# Autodesk Inventor assembly: Back_Panel_Assembly
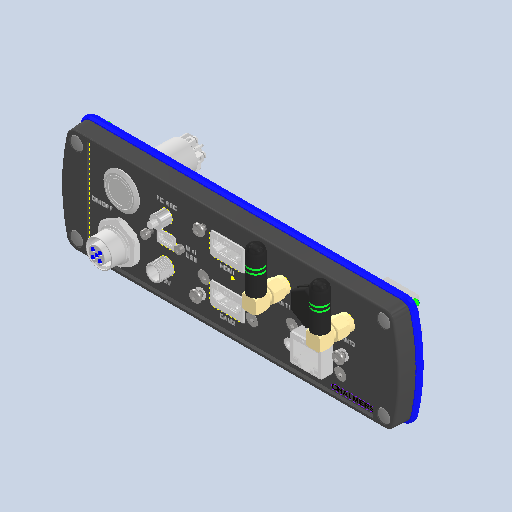
[picture p0: Inventor's stored thumbnail of the model, 512x512]
Saved by Autodesk Inventor 2022 (Build 260153000, 153)
## iProperties
Created: 2020-07-14
Part Number: Back_Panel_Assembly
Document SubType Name: Assembly
Designer: CASE-SMALL2
Author: CASE-SMALL2
## Documents named in this file (21)
- C:\Users\Viktor\Google Drive\Unicorn 2020\CAD_V2\Back_Panel\Back_Panel_Assembly.iam
- C:\Users\Viktor\Google Drive\Unicorn 2020\CAD_V2\Back_Panel\Panel\Back_Panel_Base_Assembly.iam
- C:\Users\Viktor\Google Drive\Unicorn 2020\CAD_V2\Back_Panel\Connectors\82-4551.1123\36059.iam
- C:\Users\Viktor\Google Drive\Unicorn 2020\CAD_V2\Back_Panel\Connectors\LAIRD_080-0014.ipt
- C:\Users\Viktor\Google Drive\Unicorn 2020\CAD_V2\Back_Panel\Connectors\MB2011SD3G01-CA.ipt
- C:\Users\Viktor\Google Drive\Unicorn 2020\CAD_V2\Back_Panel\Connectors\MHDRA511M0.ipt
- C:\Users\Viktor\Google Drive\Unicorn 2020\CAD_V2\Back_Panel\Connectors\M-MUSBR-B551-30.ipt
- C:\Users\Viktor\Google Drive\Unicorn 2020\CAD_V2\Back_Panel\Connectors\MRJ5784M1.ipt
- C:\Users\Viktor\Google Drive\Unicorn 2020\CAD_V2\Back_Panel\Other\PMF100585.ipt
- C:\Users\Viktor\Google Drive\Unicorn 2020\CAD_V2\Back_Panel\Other\M12_NUT_1.262.1200.50.ipt
- C:\Users\Viktor\Google Drive\Unicorn 2020\CAD_V2\Back_Panel\Connectors\ST10U.ipt
- C:\Users\Viktor\Google Drive\Unicorn 2020\CAD_V2\Back_Panel\Other\pop_PSZROX-0315.ipt
- C:\Users\Viktor\Google Drive\Unicorn 2020\CAD_V2\Back_Panel\Screws\ISO 4762 - M2 x 6ISO.ipt
- C:\Users\Viktor\Google Drive\Unicorn 2020\CAD_V2\Back_Panel\Screws\ISO 10642 - M3x6.ipt
- C:\Users\Viktor\Google Drive\Unicorn 2020\CAD_V2\Back_Panel\Screws\ISO 4762 - M3 x 4ISO.ipt
- C:\Users\Viktor\Google Drive\Unicorn 2020\CAD_V2\Back_Panel\Screws\ISO 7380-1 - M3 x 6.ipt
- C:\Users\Viktor\Google Drive\Unicorn 2020\CAD_V2\Back_Panel\Screws\ISO 7380-1 - M3 x 8.ipt
- C:\Users\Viktor\Google Drive\Unicorn 2020\CAD_V2\Back_Panel\Other\GW.26.0152\GW.26.0152_web.ipt
- C:\Users\Viktor\Google Drive\Unicorn 2020\CAD_V2\Back_Panel\Screws\ISO 4762 - M2 x 8ISO.ipt
- C:\Users\Viktor\Google Drive\Unicorn 2020\CAD_V2\Back_Panel\Connectors\c-t4131012041-000\c-t4131012041-000.ipt
- C:\Users\Viktor\Google Drive\Unicorn 2020\CAD_V2\Back_Panel\Connectors\c-t4131012041-000\M12_NUT.ipt
## Components (34 placed, 20 different names)
1. Back_Panel_Base_Assembly:1 [sub-assembly] — Rigid:1, Rigid:6, Rigid:11, Rigid:15, Rigid:16, Rigid:17, Rigid:18, Rigid:19, Rigid:21, Rigid:22, Rigid:23, Rigid:24, Rigid:25, Rigid:33, Rigid:34, Rigid:35, Rigid:36, Rigid:39, Rigid:40, Insert:1, Insert:2, Angle:1, Angle:2, Rigid:41, Rigid:42, Rigid:43, Rigid:44, Rigid:45
2. 36059:1 [sub-assembly] — Rigid:1
3. LAIRD_080-0014:1 — Rigid:45
4. LAIRD_080-0014:2 — Rigid:44
5. MB2011SD3G01-CA:1 — Rigid:34
6. MHDRA511M0:1 — Rigid:6
7. MHDRA511M0:2 — Rigid:39
8. M-MUSBR-B551-30:1 — Rigid:11
9. MRJ5784M1:1 — Rigid:40
10. PMF100585:1 — Rigid:36
11. M12_NUT_1.262.1200.50:1 — Rigid:35
12. ST10U:1 — Rigid:33
13. pop_PSZROX-0315:1 — Rigid:17, Rigid:28
14. pop_PSZROX-0315:2 — Rigid:15, Rigid:26, Rigid:31
15. pop_PSZROX-0315:3 — Rigid:16, Rigid:30
16. pop_PSZROX-0315:4 — Rigid:18, Rigid:29, Rigid:32
17. ISO 4762 - M2 x 6ISO:2 — Rigid:19
18. ISO 4762 - M2 x 8ISO:1 — Rigid:41
19. ISO 10642 - M3x6:1 — Rigid:21
20. ISO 10642 - M3x6:2 — Rigid:22
21. ISO 10642 - M3x6:3 — Rigid:23
22. ISO 10642 - M3x6:4 — Rigid:24
23. ISO 10642 - M3x6:5 — Rigid:25
24. ISO 4762 - M3 x 4ISO:1 — Rigid:30
25. ISO 4762 - M3 x 4ISO:2 — Rigid:26
26. ISO 4762 - M3 x 4ISO:3 — Rigid:28
27. ISO 4762 - M3 x 4ISO:4 — Rigid:29
28. ISO 7380-1 - M3 x 6:1 — Rigid:31
29. ISO 7380-1 - M3 x 6:2 — Rigid:32
30. ISO 7380-1 - M3 x 8:1
31. GW.26.0152_web:1 — Insert:2, Angle:2
32. GW.26.0152_web:2 — Insert:1, Angle:1
33. c-t4131012041-000:1 — Rigid:42
34. M12_NUT:1 — Rigid:43
## Relationships (34: WeldJoint 30, Insert 2, Angle 2)
- Rigid:1 [WeldJoint]: Back_Panel_Base_Assembly:1 ↔ 36059:1
- Rigid:6 [WeldJoint]: Back_Panel_Base_Assembly:1 ↔ MHDRA511M0:1
- Rigid:11 [WeldJoint]: Back_Panel_Base_Assembly:1 ↔ M-MUSBR-B551-30:1
- Rigid:15 [WeldJoint]: Back_Panel_Base_Assembly:1 ↔ pop_PSZROX-0315:2
- Rigid:16 [WeldJoint]: Back_Panel_Base_Assembly:1 ↔ pop_PSZROX-0315:3
- Rigid:17 [WeldJoint]: Back_Panel_Base_Assembly:1 ↔ pop_PSZROX-0315:1
- Rigid:18 [WeldJoint]: Back_Panel_Base_Assembly:1 ↔ pop_PSZROX-0315:4
- Rigid:19 [WeldJoint]: Back_Panel_Base_Assembly:1 ↔ ISO 4762 - M2 x 6ISO:2
- Rigid:21 [WeldJoint]: Back_Panel_Base_Assembly:1 ↔ ISO 10642 - M3x6:1
- Rigid:22 [WeldJoint]: Back_Panel_Base_Assembly:1 ↔ ISO 10642 - M3x6:2
- Rigid:23 [WeldJoint]: Back_Panel_Base_Assembly:1 ↔ ISO 10642 - M3x6:3
- Rigid:24 [WeldJoint]: Back_Panel_Base_Assembly:1 ↔ ISO 10642 - M3x6:4
- Rigid:25 [WeldJoint]: Back_Panel_Base_Assembly:1 ↔ ISO 10642 - M3x6:5
- Rigid:26 [WeldJoint] (2 mm): pop_PSZROX-0315:2 ↔ ISO 4762 - M3 x 4ISO:2
- Rigid:28 [WeldJoint] (-2 mm): pop_PSZROX-0315:1 ↔ ISO 4762 - M3 x 4ISO:3
- Rigid:29 [WeldJoint] (-2 mm): pop_PSZROX-0315:4 ↔ ISO 4762 - M3 x 4ISO:4
- Rigid:30 [WeldJoint] (-2 mm): pop_PSZROX-0315:3 ↔ ISO 4762 - M3 x 4ISO:1
- Rigid:31 [WeldJoint] (-2 mm): pop_PSZROX-0315:2 ↔ ISO 7380-1 - M3 x 6:1
- Rigid:32 [WeldJoint] (2 mm): pop_PSZROX-0315:4 ↔ ISO 7380-1 - M3 x 6:2
- Rigid:33 [WeldJoint]: Back_Panel_Base_Assembly:1 ↔ ST10U:1
- Rigid:34 [WeldJoint]: Back_Panel_Base_Assembly:1 ↔ MB2011SD3G01-CA:1
- Rigid:35 [WeldJoint]: Back_Panel_Base_Assembly:1 ↔ M12_NUT_1.262.1200.50:1
- Rigid:36 [WeldJoint]: Back_Panel_Base_Assembly:1 ↔ PMF100585:1
- Rigid:39 [WeldJoint]: Back_Panel_Base_Assembly:1 ↔ MHDRA511M0:2
- Rigid:40 [WeldJoint]: Back_Panel_Base_Assembly:1 ↔ MRJ5784M1:1
- Insert:1 (-4 mm): Back_Panel_Base_Assembly:1 ↔ GW.26.0152_web:2
- Insert:2 (-4 mm): Back_Panel_Base_Assembly:1 ↔ GW.26.0152_web:1
- Angle:1 (270 deg): Back_Panel_Base_Assembly:1 ↔ GW.26.0152_web:2
- Angle:2 (270 deg): Back_Panel_Base_Assembly:1 ↔ GW.26.0152_web:1
- Rigid:41 [WeldJoint] (-2 mm): Back_Panel_Base_Assembly:1 ↔ ISO 4762 - M2 x 8ISO:1
- Rigid:42 [WeldJoint]: Back_Panel_Base_Assembly:1 ↔ c-t4131012041-000:1
- Rigid:43 [WeldJoint]: Back_Panel_Base_Assembly:1 ↔ M12_NUT:1
- Rigid:44 [WeldJoint]: Back_Panel_Base_Assembly:1 ↔ LAIRD_080-0014:2
- Rigid:45 [WeldJoint]: Back_Panel_Base_Assembly:1 ↔ LAIRD_080-0014:1
